# Autodesk Inventor assembly: cajas_V2
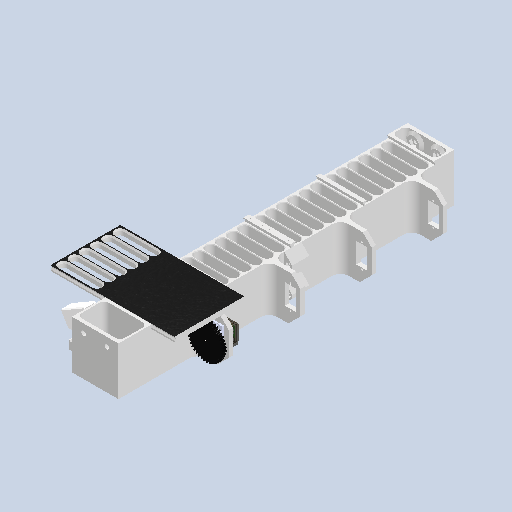
[picture p0: Inventor's stored thumbnail of the model, 512x512]
Saved by Autodesk Inventor 2022 (Build 260153000, 153)
## iProperties
Created: 2021-03-06
Part Number: cajas_V2
Document SubType Name: Assembly
Designer: juanp
Author: juanp
## Documents named in this file (6)
- C:\Users\juanp\Desktop\Robocol\EVA\V2 (Actual)\Cajas\cajas_V2.iam
- C:\Users\juanp\Desktop\Robocol\EVA\V2 (Actual)\Cajas\cajas_V2.ipt
- C:\Users\juanp\Desktop\Robocol\EVA\V2 (Actual)\Cajas\Engranaje.ipt
- C:\Users\juanp\Desktop\Robocol\EVA\V2 (Actual)\Cajas\Puerta Cremallera_V2.ipt
- C:\Users\juanp\Desktop\Robocol\EVA\Recursos\Servo MG90S\MG90S.iam
- C:\Users\juanp\Desktop\Robocol\EVA\V2 (Actual)\Cajas\Soporte motor.ipt
## Components (5 placed, 5 different names)
1. cajas_V2:1 — Mate:6, Mate:7, Mate:8, Mate:9, Mate:10, Mate:13, Angle:1
2. Engranaje:1 — Mate:11, Mate:12, Rotation/Translation:1
3. Puerta Cremallera_V2:1 — Mate:6, Mate:7, Rotation/Translation:1
4. MG90S:1 [sub-assembly] — Mate:8, Mate:9, Mate:10, Mate:11, Mate:12
5. Soporte motor:1 — Mate:13, Angle:1
## Relationships (10: Mate 8, RelateRotateTranslate 1, Angle 1)
- Mate:6: cajas_V2:1 ↔ Puerta Cremallera_V2:1
- Mate:7: cajas_V2:1 ↔ Puerta Cremallera_V2:1
- Mate:8: cajas_V2:1 ↔ MG90S:1
- Mate:9: cajas_V2:1 ↔ MG90S:1
- Mate:10: cajas_V2:1 ↔ MG90S:1
- Mate:11: Engranaje:1 ↔ MG90S:1
- Mate:12: Engranaje:1 ↔ MG90S:1
- Rotation/Translation:1 [RelateRotateTranslate] (125.664 mm): Engranaje:1 ↔ Puerta Cremallera_V2:1
- Mate:13: cajas_V2:1 ↔ Soporte motor:1
- Angle:1 (180 deg): cajas_V2:1 ↔ Soporte motor:1
